# Autodesk Inventor assembly: roller-hand-v1-P
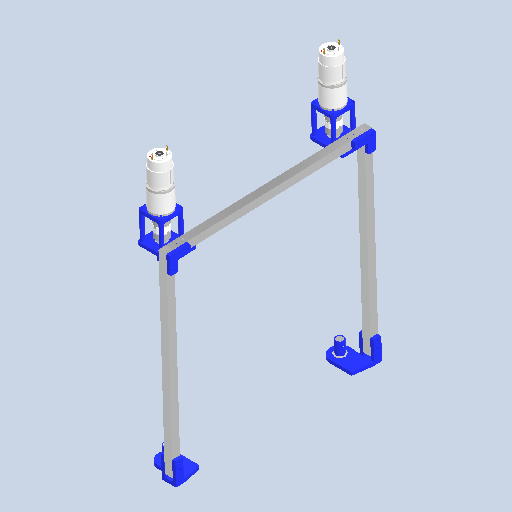
[picture p0: Inventor's stored thumbnail of the model, 512x512]
Saved by Autodesk Inventor 2025.1 (Build 291241000, 241)
## iProperties
Created: 2024-10-01
Part Number: roller-hand-v1-P
Document SubType Name: Assembly
Designer: haruy
Author: haruy
## Documents named in this file (13)
- C:\Users\haruy\Documents\ロボコン\NHK2025\cad\nagahisa\hand\roller\roller-hand-v1-P.iam
- C:\Users\haruy\Documents\ロボコン\NHK2025\cad\nagahisa\hand\roller\roller-hand-v1-3DP-bearing-m-side.ipt
- C:\Users\haruy\Documents\ロボコン\NHK2025\cad\nagahisa\hand\roller\roller-hand-v1-ASP-Base.ipt
- C:\Users\haruy\Documents\ロボコン\NHK2025\cad\000_parts\ベアリング\10\bear_10_15_sn.ipt
- C:\Users\haruy\Documents\ロボコン\NHK2025\cad\nagahisa\hand\roller\roller-hand-v1-3DP-m385-m.ipt
- C:\Users\haruy\Documents\ロボコン\NHK2025\cad\000_parts\モーター\Geared_RS-385.iam
- C:\Users\haruy\Documents\ロボコン\NHK2025\cad\nagahisa\hand\roller\MOR-20C-6-10.iam
- C:\Users\haruy\Documents\ロボコン\NHK2025\cad\nagahisa\hand\roller\roller-hand-v1-Shaft-m.ipt
- C:\Users\haruy\Documents\ロボコン\NHK2025\cad\nagahisa\hand\roller\roller-hand-v1-3DP-L-F.ipt
- C:\Users\haruy\Documents\ロボコン\NHK2025\cad\nagahisa\hand\roller\roller-hand-v1-3DP-bearing-r-side.ipt
- C:\Users\haruy\Documents\ロボコン\NHK2025\cad\nagahisa\hand\roller\roller-hand-v1-3DP-bearing-r-side_MIR.ipt
- C:\Users\haruy\Documents\ロボコン\NHK2025\cad\nagahisa\hand\roller\roller-hand-v1-Shaft-r.ipt
- C:\Users\haruy\Documents\ロボコン\NHK2025\cad\nagahisa\hand\roller\roller-hand-v1-3DP-shaft-spesa.ipt
## Components (25 placed, 12 different names)
1. roller-hand-v1-3DP-bearing-m-side:1 — 挿入:1, 挿入:2, 挿入:5, 挿入:7, 挿入:8
2. roller-hand-v1-ASP-Base:1 — 挿入:1, 挿入:2, 挿入:3, 挿入:4, 挿入:17, 挿入:18, 挿入:19, 挿入:20, 挿入:21, 挿入:22, フラッシュ:1, 挿入:24, 挿入:25
3. roller-hand-v1-3DP-bearing-m-side:2 — 挿入:3, 挿入:4, 挿入:6, 挿入:9, 挿入:10
4. bear_10_15_sn:1 — 挿入:5
5. bear_10_15_sn:2 — 挿入:6
6. roller-hand-v1-3DP-m385-m:1 — 挿入:7, 挿入:8, 挿入:11
7. roller-hand-v1-3DP-m385-m:2 — 挿入:9, 挿入:10, 挿入:12
8. Geared_RS-385:1 [sub-assembly] — 挿入:11, 挿入:13
9. Geared_RS-385:2 [sub-assembly] — 挿入:12, 挿入:14
10. MOR-20C-6-10:1 [sub-assembly] — 挿入:13, 挿入:15
11. MOR-20C-6-10:2 [sub-assembly] — 挿入:14, 挿入:16
12. roller-hand-v1-Shaft-m:1 — 挿入:15, 挿入:29
13. roller-hand-v1-Shaft-m:2 — 挿入:16, 挿入:30
14. roller-hand-v1-3DP-L-F:1 — 挿入:17, 挿入:18
15. roller-hand-v1-3DP-L-F:2 — 挿入:19, 挿入:20
16. roller-hand-v1-3DP-bearing-r-side:1 — 挿入:21, 挿入:22, 挿入:23, 挿入:27
17. bear_10_15_sn:3 — 挿入:23
18. roller-hand-v1-3DP-bearing-r-side_MIR:1 — 挿入:24, 挿入:25, 挿入:26, 挿入:28
19. bear_10_15_sn:4 — 挿入:26
20. roller-hand-v1-Shaft-r:1 — 挿入:27, 挿入:31
21. roller-hand-v1-Shaft-r:2 — 挿入:28, 挿入:32
22. roller-hand-v1-3DP-shaft-spesa:1 — 挿入:29
23. roller-hand-v1-3DP-shaft-spesa:2 — 挿入:30
24. roller-hand-v1-3DP-shaft-spesa:3 — 挿入:31
25. roller-hand-v1-3DP-shaft-spesa:4 — 挿入:32
## Relationships (33: Insert 32, Flush 1)
- 挿入:1 [Insert]: roller-hand-v1-3DP-bearing-m-side:1 ↔ roller-hand-v1-ASP-Base:1
- 挿入:2 [Insert]: roller-hand-v1-3DP-bearing-m-side:1 ↔ roller-hand-v1-ASP-Base:1
- 挿入:3 [Insert]: roller-hand-v1-ASP-Base:1 ↔ roller-hand-v1-3DP-bearing-m-side:2
- 挿入:4 [Insert]: roller-hand-v1-ASP-Base:1 ↔ roller-hand-v1-3DP-bearing-m-side:2
- 挿入:5 [Insert]: roller-hand-v1-3DP-bearing-m-side:1 ↔ bear_10_15_sn:1
- 挿入:6 [Insert]: roller-hand-v1-3DP-bearing-m-side:2 ↔ bear_10_15_sn:2
- 挿入:7 [Insert]: roller-hand-v1-3DP-bearing-m-side:1 ↔ roller-hand-v1-3DP-m385-m:1
- 挿入:8 [Insert]: roller-hand-v1-3DP-bearing-m-side:1 ↔ roller-hand-v1-3DP-m385-m:1
- 挿入:9 [Insert]: roller-hand-v1-3DP-bearing-m-side:2 ↔ roller-hand-v1-3DP-m385-m:2
- 挿入:10 [Insert]: roller-hand-v1-3DP-bearing-m-side:2 ↔ roller-hand-v1-3DP-m385-m:2
- 挿入:11 [Insert]: roller-hand-v1-3DP-m385-m:1 ↔ Geared_RS-385:1
- 挿入:12 [Insert]: roller-hand-v1-3DP-m385-m:2 ↔ Geared_RS-385:2
- 挿入:13 [Insert] (-8 mm): Geared_RS-385:1 ↔ MOR-20C-6-10:1
- 挿入:14 [Insert] (-8 mm): Geared_RS-385:2 ↔ MOR-20C-6-10:2
- 挿入:15 [Insert] (-8 mm): MOR-20C-6-10:1 ↔ roller-hand-v1-Shaft-m:1
- 挿入:16 [Insert] (-8 mm): MOR-20C-6-10:2 ↔ roller-hand-v1-Shaft-m:2
- 挿入:17 [Insert]: roller-hand-v1-ASP-Base:1 ↔ roller-hand-v1-3DP-L-F:1
- 挿入:18 [Insert]: roller-hand-v1-ASP-Base:1 ↔ roller-hand-v1-3DP-L-F:1
- 挿入:19 [Insert]: roller-hand-v1-ASP-Base:1 ↔ roller-hand-v1-3DP-L-F:2
- 挿入:20 [Insert]: roller-hand-v1-ASP-Base:1 ↔ roller-hand-v1-3DP-L-F:2
- 挿入:21 [Insert]: roller-hand-v1-ASP-Base:1 ↔ roller-hand-v1-3DP-bearing-r-side:1
- 挿入:22 [Insert]: roller-hand-v1-ASP-Base:1 ↔ roller-hand-v1-3DP-bearing-r-side:1
- 挿入:23 [Insert]: roller-hand-v1-3DP-bearing-r-side:1 ↔ bear_10_15_sn:3
- フラッシュ:1 [Flush] (-157.5 mm): roller-hand-v1-ASP-Base:1
- 挿入:24 [Insert]: roller-hand-v1-ASP-Base:1 ↔ roller-hand-v1-3DP-bearing-r-side_MIR:1
- 挿入:25 [Insert]: roller-hand-v1-ASP-Base:1 ↔ roller-hand-v1-3DP-bearing-r-side_MIR:1
- 挿入:26 [Insert]: roller-hand-v1-3DP-bearing-r-side_MIR:1 ↔ bear_10_15_sn:4
- 挿入:27 [Insert]: roller-hand-v1-3DP-bearing-r-side:1 ↔ roller-hand-v1-Shaft-r:1
- 挿入:28 [Insert]: roller-hand-v1-3DP-bearing-r-side_MIR:1 ↔ roller-hand-v1-Shaft-r:2
- 挿入:29 [Insert]: roller-hand-v1-Shaft-m:1 ↔ roller-hand-v1-3DP-shaft-spesa:1
- 挿入:30 [Insert]: roller-hand-v1-Shaft-m:2 ↔ roller-hand-v1-3DP-shaft-spesa:2
- 挿入:31 [Insert]: roller-hand-v1-Shaft-r:1 ↔ roller-hand-v1-3DP-shaft-spesa:3
- 挿入:32 [Insert]: roller-hand-v1-Shaft-r:2 ↔ roller-hand-v1-3DP-shaft-spesa:4
